# Autodesk Inventor assembly: Phone assembly solution
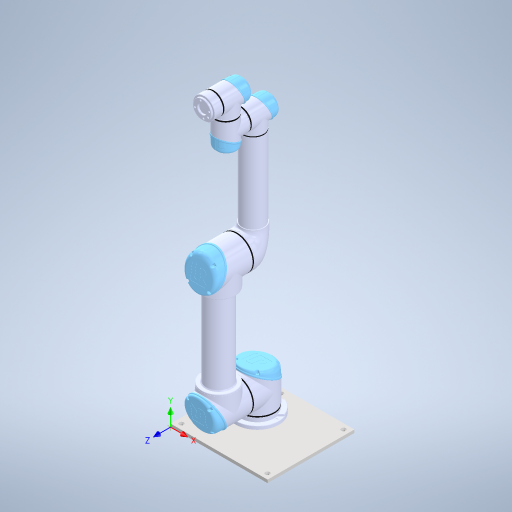
[picture p0: Inventor's stored thumbnail of the model, 512x512]
Saved by Autodesk Inventor 2024 (Build 280153000, 153)
## iProperties
Created: 2024-03-26
Part Number: Phone assembly solution
Document SubType Name: Assembly
Designer: jens1
Author: jens1
## Documents named in this file (3)
- C:\Users\jens1\Documents\GitHub\P2\3D modeller\Phone assembly solution.iam
- C:\Users\jens1\Documents\GitHub\P2\3D modeller\UR5\UR5\UR5.iam
- C:\Users\jens1\Documents\GitHub\P2\3D modeller\Mount plate UR.ipt
## Components (2 placed, 2 different names)
1. UR5:1 [sub-assembly] — Mate:2, Mate:3, Mate:4, Tangent:1
2. Mount plate UR:1 — Mate:1, Mate:2, Mate:3, Mate:4, Tangent:1
## Relationships (5: Mate 4, Tangent 1)
- Mate:1: Mount plate UR:1
- Mate:2: UR5:1 ↔ Mount plate UR:1
- Mate:3 (-116 mm): UR5:1 ↔ Mount plate UR:1
- Mate:4 (-116 mm): UR5:1 ↔ Mount plate UR:1
- Tangent:1 (0.25 mm): UR5:1 ↔ Mount plate UR:1
